# Autodesk Inventor assembly: standoff_brace_triangle
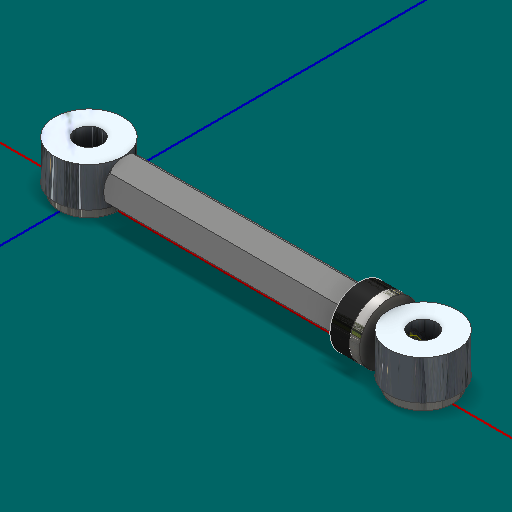
[picture p0: Inventor's stored thumbnail of the model, 512x512]
Saved by Autodesk Inventor 2025 (Build 290162000, 162)
## iProperties
Created: 2024-08-17
Part Number: standoff_brace_triangle
Document SubType Name: Assembly
Designer: averey
Author: averey
## Documents named in this file (8)
- C:\Users\avere\vex_robotics_high_stakes\hardware\cad\ATLAS\chassis\structure\standoff_brace_triangle.iam
- C:\Users\avere\vex_robotics_high_stakes\hardware\cad\VEX-CAD-Inventor\Motion\Shaft LS\Shaft Collar ipts\Shaft Collar No Screw.ipt
- C:\Users\avere\vex_robotics_high_stakes\hardware\cad\VEX-CAD-Inventor\Structure\Standoff.ipt
- C:\Users\avere\vex_robotics_high_stakes\hardware\cad\VEX-CAD-Inventor\Structure\Standoff\Standoff 1.50.ipt
- C:\Users\avere\vex_robotics_high_stakes\hardware\cad\VEX-CAD-Inventor\Motion\Spacers\Washer Steel.ipt
- C:\Users\avere\vex_robotics_high_stakes\hardware\cad\VEX-CAD-Inventor\Motion\Spacers\Washer Steel\SWasher .375 OD x .062500.ipt
- C:\Users\avere\vex_robotics_high_stakes\hardware\cad\VEX-CAD-Inventor\Motion\Spacers\Spacer Nylon .375 OD\NSpacer .375 OD x .125.ipt
- C:\Users\avere\vex_robotics_high_stakes\hardware\cad\VEX-CAD-Inventor\Motion\Spacers\Spacer Nylon .375 OD.ipt
## Components (7 placed, 4 different names)
1. Shaft Collar No Screw:1 — Mate:2, Angle:2, Insert:7, Insert:12
2. Shaft Collar No Screw:2 — Angle:3, Insert:6, Insert:11, Insert:12
3. SWasher .375 OD x .062500:3 — Insert:6
4. SWasher .375 OD x .062500:4 — Insert:7
5. NSpacer .375 OD x .125:1 — Insert:8, Insert:10
6. SWasher .375 OD x .062500:5 — Insert:8, Insert:11
7. Standoff 1.50:1 — Insert:10
## Relationships (10: Insert 6, Mate 2, Angle 2)
- [Mate]: Shaft Collar No Screw:1 ↔ Shaft Collar No Screw:2
- Mate:2: Shaft Collar No Screw:1
- Angle:2 (0 deg): Shaft Collar No Screw:1
- Angle:3 (0 deg): Shaft Collar No Screw:2
- Insert:6: Shaft Collar No Screw:2 ↔ SWasher .375 OD x .062500:3
- Insert:7: Shaft Collar No Screw:1 ↔ SWasher .375 OD x .062500:4
- Insert:8: NSpacer .375 OD x .125:1 ↔ SWasher .375 OD x .062500:5
- Insert:10: NSpacer .375 OD x .125:1 ↔ Standoff 1.50:1
- Insert:11: Shaft Collar No Screw:2 ↔ SWasher .375 OD x .062500:5
- Insert:12 (42.8815 mm): Shaft Collar No Screw:1 ↔ Shaft Collar No Screw:2
